# Autodesk Inventor assembly: MG-Raendelmutter M4
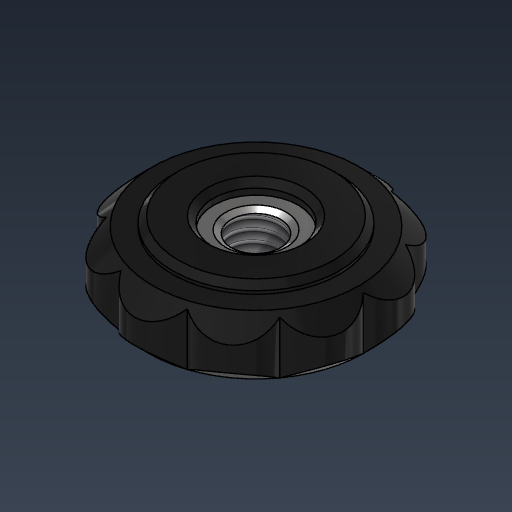
[picture p0: Inventor's stored thumbnail of the model, 512x512]
Saved by Autodesk Inventor 2023.1 (Build 271208000, 208)
## iProperties
Part Number: MG-Raendelmutter M4
Material: Generisch
Document SubType Name: Assembly
Designer: rYan
Author: rYan
## Documents named in this file (3)
- D:\TIGERsGIT\Hardware\mechanik\2024\Inventor\Robot\Case\MG-Raendelmutter M4.iam
- D:\TIGERsGIT\Hardware\mechanik\2024\Inventor\Robot\Case\Raendelmutter M4 Druckteil.ipt
- D:\TIGERsGIT\Hardware\mechanik\2024\Inventor\Inhaltscenter\de-DE\DIN 934\DIN 934 - M4 x 0,7.ipt
## Components (2 placed, 2 different names)
1. Raendelmutter M4 Druckteil:1 — Fluchtend:1, Fluchtend:2, Fluchtend:3, Passend:5, Passend:1, Winkel:1
2. DIN 934 - ersetzt durch DIN EN 24032/28673/28674 M4:1 — Passend:5, Passend:1, Winkel:1
## Relationships (6: Flush 3, Mate 2, Angle 1)
- Fluchtend:1 [Flush]: Raendelmutter M4 Druckteil:1
- Fluchtend:2 [Flush]: Raendelmutter M4 Druckteil:1
- Fluchtend:3 [Flush]: Raendelmutter M4 Druckteil:1
- Passend:5 [Mate]: Raendelmutter M4 Druckteil:1 ↔ DIN 934 - ersetzt durch DIN EN 24032/28673/28674 M4:1
- Passend:1 [Mate]: Raendelmutter M4 Druckteil:1 ↔ DIN 934 - ersetzt durch DIN EN 24032/28673/28674 M4:1
- Winkel:1 [Angle] (0 deg): Raendelmutter M4 Druckteil:1 ↔ DIN 934 - ersetzt durch DIN EN 24032/28673/28674 M4:1
